# Autodesk Inventor assembly: assembly_carWithRoofBar
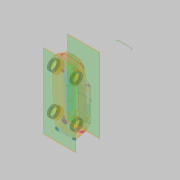
[picture p0: Inventor's stored thumbnail of the model, 180x180]
Saved by Autodesk Inventor 2021 (Build 250183000, 183)
## iProperties
Created: 2021-05-31
Part Number: assembly_carWithRoofBar
Document SubType Name: Assembly
Designer: Watchdog
Author: Watchdog
## Documents named in this file (3)
- C:\Users\Watchdog\OneDrive - Flinders\Advn Mech Design Shared\6_Development\2_Design\inventor\vehicle_wheelchair\assembly_carWithRoofBar.iam
- C:\Users\Watchdog\OneDrive - Flinders\Advn Mech Design Shared\6_Development\2_Design\inventor\vehicle_wheelchair\mb_gls\ext_GLS Assembly.iam
- C:\Users\Watchdog\OneDrive - Flinders\Advn Mech Design Shared\6_Development\2_Design\inventor\support\roof_bar\ext_roof bar assembly.iam
## Components (3 placed, 2 different names)
1. ext_GLS Assembly:1 [sub-assembly] — Flush:1, Flush:2, Flush:3, Angle:1, Angle:2
2. ext_roof bar assembly:1 [sub-assembly]
3. ext_roof bar assembly:2 [sub-assembly] — Angle:1, Angle:2
## Relationships (5: Flush 3, Angle 2)
- Flush:1: ext_GLS Assembly:1
- Flush:2: ext_GLS Assembly:1
- Flush:3: ext_GLS Assembly:1
- Angle:1 (0 deg): ext_GLS Assembly:1 ↔ ext_roof bar assembly:2
- Angle:2 (180 deg): ext_GLS Assembly:1 ↔ ext_roof bar assembly:2
